# Autodesk Inventor assembly: Engine Assembly
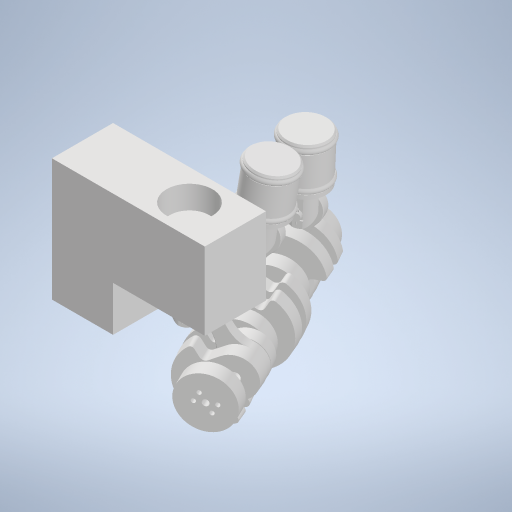
[picture p0: Inventor's stored thumbnail of the model, 512x512]
Saved by Autodesk Inventor 2023 (Build 270158000, 158)
## iProperties
Created: 2023-01-04
Part Number: Engine Assembly
Document SubType Name: Assembly
Designer: tgr41
Author: tgr41
## Documents named in this file (7)
- C:\Users\tommy\Documents\Repositories\Steam-Engine\1.5x1 Inch 3 Cylidner\Cast and Assembled V5\Engine Assembly.iam
- C:\Users\tommy\Documents\Repositories\Steam-Engine\1.5x1 Inch 3 Cylidner\Cast and Assembled V5\A.Crankshaft Subassembly.iam
- C:\Users\tommy\Documents\Repositories\Steam-Engine\1.5x1 Inch 3 Cylidner\Cast and Assembled V5\A.Piston Subassembly.iam
- C:\Users\tommy\Documents\Repositories\Steam-Engine\1.5x1 Inch 3 Cylidner\Cast and Assembled V5\C.Connecting Rod.ipt
- C:\Users\tommy\Documents\Repositories\Steam-Engine\1.5x1 Inch 3 Cylidner\Cast and Assembled V5\C.Crank Connect Shaft.ipt
- C:\Users\tommy\Documents\Repositories\Steam-Engine\1.5x1 Inch 3 Cylidner\Cast and Assembled V5\C.Crankshaft Main Bearing.ipt
- C:\Users\tommy\Documents\Repositories\Steam-Engine\1.5x1 Inch 3 Cylidner\Cast and Assembled V5\E.Cylinder Block.ipt
## Components (10 placed, 6 different names)
1. A.Crankshaft Subassembly:1 [sub-assembly] — Mate:4, Mate:5, Mate:6, Mate:8, Mate:9, Mate:10, Mate:11, Mate:12, Mate:16
2. A.Piston Subassembly:1 [sub-assembly] — Mate:1
3. C.Connecting Rod:1 — Mate:1, Mate:4, Mate:9
4. A.Piston Subassembly:2 [sub-assembly]
5. C.Connecting Rod:2 — Mate:5, Mate:8
6. A.Piston Subassembly:3 [sub-assembly] — Mate:17
7. C.Connecting Rod:3 — Mate:6, Mate:16
8. C.Crank Connect Shaft:1 — Mate:10, Mate:11, Mate:12, Mate:13, Flush:1
9. C.Crankshaft Main Bearing:1 — Mate:13, Flush:1
10. E.Cylinder Block:2 — Mate:17
## Relationships (15: Mate 14, Flush 1)
- Mate:1: A.Piston Subassembly:1 ↔ C.Connecting Rod:1
- [Mate]: A.Piston Subassembly:2 ↔ C.Connecting Rod:2
- [Mate]: A.Piston Subassembly:3 ↔ C.Connecting Rod:3
- Mate:4: A.Crankshaft Subassembly:1 ↔ C.Connecting Rod:1
- Mate:5: A.Crankshaft Subassembly:1 ↔ C.Connecting Rod:2
- Mate:6: A.Crankshaft Subassembly:1 ↔ C.Connecting Rod:3
- Mate:8: A.Crankshaft Subassembly:1 ↔ C.Connecting Rod:2
- Mate:9: A.Crankshaft Subassembly:1 ↔ C.Connecting Rod:1
- Mate:10: A.Crankshaft Subassembly:1 ↔ C.Crank Connect Shaft:1
- Mate:11: A.Crankshaft Subassembly:1 ↔ C.Crank Connect Shaft:1
- Mate:12: A.Crankshaft Subassembly:1 ↔ C.Crank Connect Shaft:1
- Mate:13: C.Crank Connect Shaft:1 ↔ C.Crankshaft Main Bearing:1
- Flush:1: C.Crank Connect Shaft:1 ↔ C.Crankshaft Main Bearing:1
- Mate:16: A.Crankshaft Subassembly:1 ↔ C.Connecting Rod:3
- Mate:17: A.Piston Subassembly:3 ↔ E.Cylinder Block:2
## Named parameters: d1_d0 = 0 mm, d2_d0 = 0 mm
